# Autodesk Inventor assembly: DraftAssembly
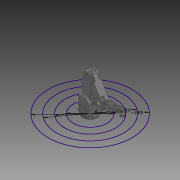
[picture p0: Inventor's stored thumbnail of the model, 180x180]
Saved by Autodesk Inventor 2020 (Build 240168000, 168)
## iProperties
Created: 2021-03-19
Part Number: DraftAssembly
Document SubType Name: Assembly
Designer: DDeGo
Author: DDeGo
## Documents named in this file (23)
- C:\Users\DDeGo\Documents\Drew\Projects\OS-ARM\cad\FirstDraft\DraftAssembly.iam
- C:\Users\DDeGo\Documents\Drew\Projects\OS-ARM\cad\FirstDraft\Base.ipt
- C:\Users\DDeGo\Documents\Drew\Projects\OS-ARM\cad\FirstDraft\Link1.ipt
- C:\Users\DDeGo\Documents\Drew\Projects\OS-ARM\cad\FirstDraft\Link2.ipt
- C:\Users\DDeGo\Documents\Drew\Projects\OS-ARM\cad\FirstDraft\CamBracket.ipt
- C:\Users\DDeGo\Documents\Drew\Projects\OS-ARM\cad\FirstDraft\Wrist.ipt
- C:\Users\DDeGo\Documents\Drew\Projects\OS-ARM\cad\FirstDraft\J1_Base.ipt
- C:\Users\DDeGo\Documents\Drew\Projects\OS-ARM\cad\FirstDraft\Link3.ipt
- C:\Users\DDeGo\Documents\Drew\Projects\OS-ARM\cad\OTS\NEMA 23 - 41mm.ipt
- C:\Users\DDeGo\Documents\Drew\Projects\OS-ARM\cad\HarmonicDrive75mm\HarmonicDrive75mm.iam
- C:\Users\DDeGo\Documents\Drew\Projects\OS-ARM\cad\OTS\6815 bearing.ipt
- C:\Users\DDeGo\Documents\Drew\Projects\OS-ARM\cad\OTS\Nema 17 22mm.ipt
- C:\Users\DDeGo\Documents\Drew\Projects\OS-ARM\cad\FirstDraft\J0_BaseMotorMount.ipt
- C:\Users\DDeGo\Documents\Drew\Projects\OS-ARM\cad\OTS\608 bearing.ipt
- C:\Users\DDeGo\Documents\Drew\Projects\OS-ARM\cad\OTS\AXK7095 thrust bearing.ipt
- C:\Users\DDeGo\Documents\Drew\Projects\OS-ARM\cad\FirstDraft\J0_BaseMotorMount2.ipt
- C:\Users\DDeGo\Documents\Drew\Projects\OS-ARM\cad\FirstDraft\J0_DriveDisc.ipt
- C:\Users\DDeGo\Documents\Drew\Projects\OS-ARM\cad\FirstDraft\J1_NewBase.ipt
- C:\Users\DDeGo\Documents\Drew\Projects\OS-ARM\cad\OTS\40mmFan.ipt
- C:\Users\DDeGo\Documents\Drew\Projects\OS-ARM\cad\OTS\6810 bearing.ipt
- C:\Users\DDeGo\Documents\Drew\Projects\OS-ARM\cad\FirstDraft\J1_NewBaseHDSide.ipt
- C:\Users\DDeGo\Documents\Drew\Projects\OS-ARM\cad\FirstDraft\EncoderV1\SmallEncoder.ipt
- C:\Users\DDeGo\Documents\Drew\Projects\OS-ARM\cad\FirstDraft\MotherboardV1\MotherboardV1.ipt
## Components (29 placed, 22 different names)
1. Base:1 — Mate:57, Mate:87, Flush:11, Flush:12, Flush:13, Mate:106, Mate:107, Mate:109, Angle:1
2. Link1:1 — Mate:30, Mate:33, Mate:34, Mate:35, Mate:49, Mate:93, Mate:94, Mate:95
3. Link2:1 — Mate:23, Mate:24, Mate:36, Mate:37, Mate:38, Flush:5, Flush:6, Flush:7, Flush:8, Flush:9, Flush:10
4. CamBracket:1 — Mate:9, Mate:12
5. Wrist:1 — Mate:9, Mate:12, Mate:25, Mate:26
6. J1_Base:1 — Mate:47, Mate:48, Mate:80, Mate:81, Mate:82, Mate:92, Mate:96, Mate:97, Mate:98, Mate:99, Mate:101, Mate:102, Mate:103, Mate:113, Mate:118, Mate:119, Mate:120
7. Link3:1 — Mate:23, Mate:24, Mate:25, Mate:26, Angle:1
8. NEMA 23 - 41mm:1 — Mate:30, Mate:49
9. HarmonicDrive75mm:1 [sub-assembly] — Mate:31, Mate:32, Mate:35, Mate:36, Mate:37, Mate:38
10. 6815 bearing:1 — Mate:31, Mate:32, Mate:33, Mate:34
11. NEMA 23 - 41mm:2 — Mate:47, Mate:48, Mate:100, Angle:2
12. NEMA 23 - 41mm:3 — Mate:77, Mate:78, Mate:79, Mate:100
13. Nema 17 22mm:1 — Flush:5, Flush:6, Flush:7
14. Nema 17 22mm:2 — Flush:8, Flush:9, Flush:10
15. J0_BaseMotorMount:1 — Mate:57, Mate:66, Mate:67, Mate:73, Mate:74, Mate:98, Mate:99, Mate:110
16. 608 bearing:1 — Mate:104, Mate:105, Mate:117
17. AXK7095 thrust bearing:1 — Mate:66, Mate:67, Mate:83, Mate:84
18. J0_BaseMotorMount2:1 — Mate:73, Mate:74, Mate:77, Mate:78, Mate:79, Mate:80, Mate:81, Mate:82, Mate:104, Mate:105, Mate:116
19. J0_DriveDisc:1 — Mate:83, Mate:84, Mate:87, Mate:108
20. J1_NewBase:1 — Mate:92, Mate:96, Mate:97, Mate:114, Mate:115
21. 6815 bearing:3 — Mate:88, Mate:90, Mate:111, Mate:112
22. HarmonicDrive75mm:2 [sub-assembly] — Mate:88, Mate:90, Mate:93, Mate:94, Mate:95
23. 40mmFan:1 — Mate:101, Mate:102, Mate:103
24. 6810 bearing:1 — Mate:106, Mate:108
25. AXK7095 thrust bearing:2 — Mate:107, Mate:109, Mate:110
26. J1_NewBaseHDSide:1 — Mate:111, Mate:112, Mate:113, Mate:114, Mate:115
27. SmallEncoder:1 — Mate:116, Angle:2, Mate:117
28. SmallEncoder:2
29. MotherboardV1:1 — Mate:118, Mate:119, Mate:120
## Relationships (74: Mate 63, Flush 9, Angle 2)
- Mate:9: CamBracket:1 ↔ Wrist:1
- Mate:12: CamBracket:1 ↔ Wrist:1
- Mate:23: Link2:1 ↔ Link3:1
- Mate:24: Link2:1 ↔ Link3:1
- Mate:25: Wrist:1 ↔ Link3:1
- Mate:26: Wrist:1 ↔ Link3:1
- Mate:30 (5 mm): Link1:1 ↔ NEMA 23 - 41mm:1
- Mate:31: HarmonicDrive75mm:1 ↔ 6815 bearing:1
- Mate:32: HarmonicDrive75mm:1 ↔ 6815 bearing:1
- Mate:33: Link1:1 ↔ 6815 bearing:1
- Mate:34: Link1:1 ↔ 6815 bearing:1
- Mate:35: Link1:1 ↔ HarmonicDrive75mm:1
- Mate:36: Link2:1 ↔ HarmonicDrive75mm:1
- Mate:37: Link2:1 ↔ HarmonicDrive75mm:1
- Mate:38: Link2:1 ↔ HarmonicDrive75mm:1
- Mate:47: J1_Base:1 ↔ NEMA 23 - 41mm:2
- Mate:48 (25 mm): J1_Base:1 ↔ NEMA 23 - 41mm:2
- Mate:49: Link1:1 ↔ NEMA 23 - 41mm:1
- Flush:5 (-25 mm): Link2:1 ↔ Nema 17 22mm:1
- Flush:6 (-3 mm): Link2:1 ↔ Nema 17 22mm:1
- Flush:7 (100 mm): Link2:1 ↔ Nema 17 22mm:1
- Flush:8 (-45 mm): Link2:1 ↔ Nema 17 22mm:2
- Flush:9 (55 mm): Link2:1 ↔ Nema 17 22mm:2
- Flush:10 (-25 mm): Link2:1 ↔ Nema 17 22mm:2
- Mate:57: Base:1 ↔ J0_BaseMotorMount:1
- Mate:66: J0_BaseMotorMount:1 ↔ AXK7095 thrust bearing:1
- Mate:67: J0_BaseMotorMount:1 ↔ AXK7095 thrust bearing:1
- Mate:73: J0_BaseMotorMount:1 ↔ J0_BaseMotorMount2:1
- Mate:74: J0_BaseMotorMount:1 ↔ J0_BaseMotorMount2:1
- Mate:77: NEMA 23 - 41mm:3 ↔ J0_BaseMotorMount2:1
- Mate:78: NEMA 23 - 41mm:3 ↔ J0_BaseMotorMount2:1
- Mate:79: NEMA 23 - 41mm:3 ↔ J0_BaseMotorMount2:1
- Mate:80: J1_Base:1 ↔ J0_BaseMotorMount2:1
- Mate:81: J1_Base:1 ↔ J0_BaseMotorMount2:1
- Mate:82: J1_Base:1 ↔ J0_BaseMotorMount2:1
- Mate:83: AXK7095 thrust bearing:1 ↔ J0_DriveDisc:1
- Mate:84: AXK7095 thrust bearing:1 ↔ J0_DriveDisc:1
- Mate:87: Base:1 ↔ J0_DriveDisc:1
- Mate:88: 6815 bearing:3 ↔ HarmonicDrive75mm:2
- Mate:90: 6815 bearing:3 ↔ HarmonicDrive75mm:2
- Mate:92: J1_Base:1 ↔ J1_NewBase:1
- Mate:93: Link1:1 ↔ HarmonicDrive75mm:2
- Mate:94: Link1:1 ↔ HarmonicDrive75mm:2
- Mate:95: Link1:1 ↔ HarmonicDrive75mm:2
- Mate:96: J1_Base:1 ↔ J1_NewBase:1
- Mate:97: J1_Base:1 ↔ J1_NewBase:1
- Mate:98: J1_Base:1 ↔ J0_BaseMotorMount:1
- Mate:99: J1_Base:1 ↔ J0_BaseMotorMount:1
- Mate:100 (1 mm): NEMA 23 - 41mm:2 ↔ NEMA 23 - 41mm:3
- Flush:11: Base:1
- Flush:12: Base:1
- Flush:13: Base:1
- Mate:101: J1_Base:1 ↔ 40mmFan:1
- Mate:102: J1_Base:1 ↔ 40mmFan:1
- Mate:103: J1_Base:1 ↔ 40mmFan:1
- Mate:104: 608 bearing:1 ↔ J0_BaseMotorMount2:1
- Mate:105: 608 bearing:1 ↔ J0_BaseMotorMount2:1
- Mate:106: Base:1 ↔ 6810 bearing:1
- Mate:107: Base:1 ↔ AXK7095 thrust bearing:2
- Mate:108: J0_DriveDisc:1 ↔ 6810 bearing:1
- Mate:109: Base:1 ↔ AXK7095 thrust bearing:2
- Mate:110: J0_BaseMotorMount:1 ↔ AXK7095 thrust bearing:2
- Angle:1 (0 deg): Base:1 ↔ Link3:1
- Mate:111: 6815 bearing:3 ↔ J1_NewBaseHDSide:1
- Mate:112: 6815 bearing:3 ↔ J1_NewBaseHDSide:1
- Mate:113: J1_Base:1 ↔ J1_NewBaseHDSide:1
- Mate:114: J1_NewBase:1 ↔ J1_NewBaseHDSide:1
- Mate:115: J1_NewBase:1 ↔ J1_NewBaseHDSide:1
- Mate:116 (10 mm): J0_BaseMotorMount2:1 ↔ SmallEncoder:1
- Angle:2 (180 deg): NEMA 23 - 41mm:2 ↔ SmallEncoder:1
- Mate:117: 608 bearing:1 ↔ SmallEncoder:1
- Mate:118 (5 mm): J1_Base:1 ↔ MotherboardV1:1
- Mate:119 (12 mm): J1_Base:1 ↔ MotherboardV1:1
- Mate:120 (30 mm): J1_Base:1 ↔ MotherboardV1:1
